# Autodesk Inventor assembly: defualt_arm_assembly
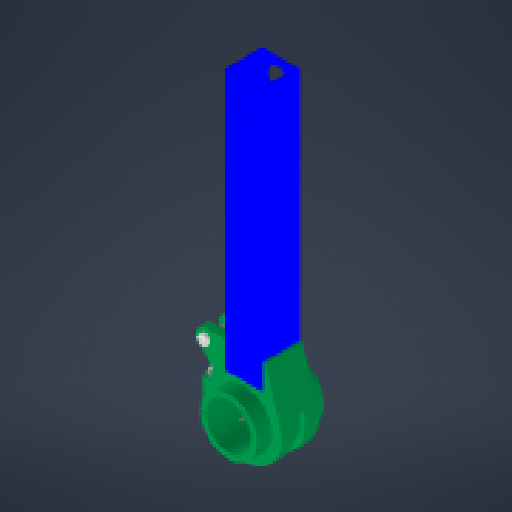
[picture p0: Inventor's stored thumbnail of the model, 512x512]
Saved by Autodesk Inventor 2024 (Build 280153000, 153)
## iProperties
Created: 2023-09-26
Part Number: defualt_arm_assembly
Document SubType Name: Assembly
Designer: user
Author: user
## Documents named in this file (6)
- D:\Docs\Robot\3d_v2\machine_body\arm_assembly\defualt_arm_assembly.iam
- D:\Docs\Robot\3d_v2\base\arm.ipt
- D:\Docs\Robot\3d_v2\machine_body\arm_assembly\motor_holder.ipt
- C:\Users\user\Documents\Inventor\Content Center Files\R2024\ru-RU\DIN 7985 (H)\DIN 7985 (H) - M3x22-H.ipt
- C:\Users\user\Documents\Inventor\Content Center Files\R2024\ru-RU\DIN 6924\DIN 6924 - M3 x 0,5.ipt
- C:\Users\user\Documents\Inventor\Content Center Files\R2024\ru-RU\DIN 7985 (H)\DIN 7985 (H) - M3x18-H.ipt
## Components (8 placed, 5 different names)
1. arm:1 — Совмещение:1, Совмещение:2, Совмещение:3, Совмещение:4, Совмещение:5, Совмещение:6
2. motor_holder:1 — Совмещение:4, Совмещение:5, Совмещение:6, Совмещение:17, Совмещение:18, Совмещение:19, Совмещение:20, Совмещение:21, Совмещение:22, Совмещение:23, Совмещение:24, Совмещение:25, Совмещение:26, Совмещение:27, Совмещение:28
3. DIN 7985 (H) M3x22-H:3 — Совмещение:17, Совмещение:18
4. DIN 6924 - заменено на DIN EN ISO 7040/10512 M3:3 — Совмещение:19, Совмещение:20
5. DIN 7985 (H) M3x18-H:1 — Совмещение:21, Совмещение:22
6. DIN 6924 - заменено на DIN EN ISO 7040/10512 M3:4 — Совмещение:23, Совмещение:24
7. DIN 7985 (H) M3x18-H:2 — Совмещение:25, Совмещение:26
8. DIN 6924 - заменено на DIN EN ISO 7040/10512 M3:5 — Совмещение:27, Совмещение:28
## Relationships (18: Mate 18)
- Совмещение:1 [Mate]: arm:1
- Совмещение:2 [Mate]: arm:1
- Совмещение:3 [Mate]: arm:1
- Совмещение:4 [Mate]: arm:1 ↔ motor_holder:1
- Совмещение:5 [Mate]: arm:1 ↔ motor_holder:1
- Совмещение:6 [Mate]: arm:1 ↔ motor_holder:1
- Совмещение:17 [Mate]: motor_holder:1 ↔ DIN 7985 (H) M3x22-H:3
- Совмещение:18 [Mate]: motor_holder:1 ↔ DIN 7985 (H) M3x22-H:3
- Совмещение:19 [Mate]: motor_holder:1 ↔ DIN 6924 - заменено на DIN EN ISO 7040/10512 M3:3
- Совмещение:20 [Mate]: motor_holder:1 ↔ DIN 6924 - заменено на DIN EN ISO 7040/10512 M3:3
- Совмещение:21 [Mate]: motor_holder:1 ↔ DIN 7985 (H) M3x18-H:1
- Совмещение:22 [Mate]: motor_holder:1 ↔ DIN 7985 (H) M3x18-H:1
- Совмещение:23 [Mate]: motor_holder:1 ↔ DIN 6924 - заменено на DIN EN ISO 7040/10512 M3:4
- Совмещение:24 [Mate]: motor_holder:1 ↔ DIN 6924 - заменено на DIN EN ISO 7040/10512 M3:4
- Совмещение:25 [Mate]: motor_holder:1 ↔ DIN 7985 (H) M3x18-H:2
- Совмещение:26 [Mate]: motor_holder:1 ↔ DIN 7985 (H) M3x18-H:2
- Совмещение:27 [Mate]: motor_holder:1 ↔ DIN 6924 - заменено на DIN EN ISO 7040/10512 M3:5
- Совмещение:28 [Mate]: motor_holder:1 ↔ DIN 6924 - заменено на DIN EN ISO 7040/10512 M3:5
